# Autodesk Inventor assembly: ASY 000 ДМФ Disk Micro filter v3.0
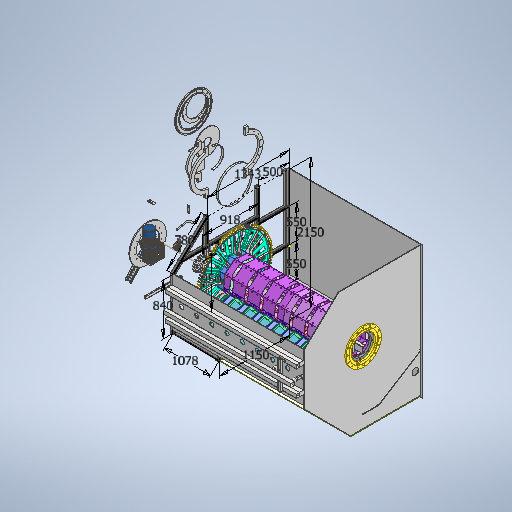
[picture p0: Inventor's stored thumbnail of the model, 512x512]
Saved by Autodesk Inventor 2026.2 (Build 302298000, 298)
## iProperties
Part Number: ASY 000 ДМФ Disk Micro filter v3.0
Document SubType Name: Assembly
Designer: admin
Author: admin
## Documents named in this file (43)
- C:\Users\admin\Documents\Inventor\DMF-Disk-Micro-Filter\ASY 000 ДМФ Disk Micro filter v3.0.iam
- C:\Users\admin\Documents\Inventor\DMF-Disk-Micro-Filter\Wall right v2.0.ipt
- C:\Users\admin\Documents\Inventor\DMF-Disk-Micro-Filter\DF1.03 Wall bottom v2.0.ipt
- C:\Users\admin\Documents\Inventor\DMF-Disk-Micro-Filter\DF1.04 Wall face v2.0.ipt
- C:\Users\admin\Documents\Inventor\DMF-Disk-Micro-Filter\ДМФ 021 кольцо прижимное нос v2.0.ipt
- C:\Users\admin\Documents\Inventor\DMF-Disk-Micro-Filter\ДМФ 032 крышка Нос v2.0.ipt
- C:\Users\admin\Documents\Inventor\DMF-Disk-Micro-Filter\ДМФ 091 Постель НОС v2.0.ipt
- C:\Users\admin\Documents\Inventor\DMF-Disk-Micro-Filter\ДМФ 022 кольцо прижимное корма v2.0.ipt
- C:\Users\admin\Documents\Inventor\DMF-Disk-Micro-Filter\ДМФ 093 Постель КОРМА v2.0.ipt
- C:\Users\admin\Documents\Inventor\DMF-Disk-Micro-Filter\ДМФ 092 Коромысло КОРМА v2.0.ipt
- C:\Users\admin\Documents\Inventor\DMF-Disk-Micro-Filter\ДМФ 055 труба илоотвода v2.0.ipt
- C:\Users\admin\Documents\Inventor\DMF-Disk-Micro-Filter\ДМФ 033 держатель лотка v2.0.ipt
- C:\Users\admin\Documents\Inventor\DMF-Disk-Micro-Filter\ASY ДМФ лоток 050 илоотвод v2.0.iam
- C:\Users\admin\Documents\Inventor\DMF-Disk-Micro-Filter\ДМФ 092 Коромысло НОС v2.0.ipt
- C:\Users\admin\Documents\Inventor\DMF-Disk-Micro-Filter\ДМФ 066 Гребенка v2.0.ipt
- C:\Users\admin\Documents\Inventor\DMF-Disk-Micro-Filter\ДМФ 025 кольцо прижимное корма наружное v2.0.ipt
- C:\Users\admin\Documents\Inventor\DMF-Disk-Micro-Filter\ДМФ 067 крышка v2.0.ipt
- C:\Users\admin\Documents\Inventor\DMF-Disk-Micro-Filter\ДМФ 081 труба форсунки v2.0.ipt
- C:\Users\admin\Documents\Inventor\DMF-Disk-Micro-Filter\ASY Обрешетка лицевая стенка.iam
- C:\Users\admin\Documents\Inventor\DMF-Disk-Micro-Filter\Вал ведущей шестерни.ipt
- C:\Users\admin\Documents\Inventor\DMF-Disk-Micro-Filter\Корпусный подшипник D35.ipt
- C:\Users\admin\Documents\Inventor\DMF-Disk-Micro-Filter\Мотор-редуктор NMRV 090(80B5).ipt
- C:\Users\admin\Documents\Inventor\DMF-Disk-Micro-Filter\DMF pancake.ipt
- C:\Users\admin\Documents\Inventor\DMF-Disk-Micro-Filter\Нога для постели.ipt
- C:\Users\admin\Documents\Inventor\DMF-Disk-Micro-Filter\Нога для постели №2.ipt
- C:\Users\admin\Documents\Inventor\DMF-Disk-Micro-Filter\ДМФ 092 Постель НОС v2.0.ipt
- C:\Users\admin\Documents\Inventor\DMF-Disk-Micro-Filter\ДМФ 094 Постель НОС крепление v2.0.ipt
- C:\Users\admin\Documents\Inventor\DMF-Disk-Micro-Filter\DMF Hat 2.0.ipt
- C:\Users\admin\Documents\Inventor\DMF-Disk-Micro-Filter\DMF Flange exit 2.0.ipt
- C:\Users\admin\Documents\Inventor\DMF-Disk-Micro-Filter\Барабан v2.1\ASY ДМФ 0100 Барабан v2.1.iam
- C:\Users\admin\Documents\Inventor\DMF-Disk-Micro-Filter\Барабан v2.1\DMF flange small gear.ipt
- C:\Users\admin\Documents\Inventor\DMF-Disk-Micro-Filter\Барабан v2.1\DMF small gear.ipt
- C:\Users\admin\Documents\Inventor\DMF-Disk-Micro-Filter\DMF Support ring tail.ipt
- C:\Users\admin\Documents\Inventor\DMF-Disk-Micro-Filter\DMF 082 коллектор болванка.ipt
- C:\Users\admin\Documents\Inventor\DMF-Disk-Micro-Filter\Барабан v2.1\DMF 2.1 Пластина паза маленькая.ipt
- C:\Users\admin\Documents\Inventor\DMF-Disk-Micro-Filter\Барабан v2.1\DMF 01 12 Барабан усилитель v2.1.ipt
- C:\Users\admin\Documents\Inventor\DMF-Disk-Micro-Filter\Барабан v2.1\DMF 2.1 01 45 Gear ring 5.ipt
- C:\Users\admin\Documents\Inventor\DMF-Disk-Micro-Filter\Барабан v2.1\DMF 2.1 01 46 Gear axis wheel 6.ipt
- C:\Users\admin\Documents\Inventor\DMF-Disk-Micro-Filter\Барабан v2.1\DMF 01 13 Барабан усилитель v2.1.ipt
- C:\Users\admin\Documents\Inventor\DMF-Disk-Micro-Filter\ДМФ 01 12 Барабан усилитель.ipt
- C:\Users\admin\Documents\Inventor\DMF-Disk-Micro-Filter\ДМФ 01 15 Барабан усилитель борта.ipt
- C:\Users\admin\Documents\Inventor\DMF-Disk-Micro-Filter\ДМФ 01 15 Барабан усилитель борта_CPY.ipt
- C:\Users\admin\Documents\Inventor\DMF-Disk-Micro-Filter\Барабан v2.1\DMF flange small gear 2.ipt
## Components (43 placed, 42 different names)
1. Wall right v2.0:1
2. DF1.03 Wall bottom v2.0:1
3. DF1.04 Wall face v2.0:1
4. ДМФ 021 кольцо прижимное нос v2.0:1
5. ДМФ 032 крышка Нос v2.0:1
6. ДМФ 091 Постель НОС v2.0:1
7. ДМФ 022 кольцо прижимное корма v2.0:1
8. ДМФ 093 Постель КОРМА v2.0:1
9. Постель 204 корма:1
10. ДМФ 055 труба илоотвода v2.0:1
11. ДМФ 033 держатель лотка v2.0:1
12. ASY ДМФ лоток 050 илоотвод v2.0:1 [sub-assembly]
13. ДМФ 092 Коромысло НОС v2.0:1
14. ДМФ 066 Гребенка v2.0:1
15. ДМФ 025 кольцо прижимное корма наружное v2.0:1
16. ДМФ 067 крышка v2.0:1
17. ДМФ 081 труба форсунки v2.0:1
18. ASY Обрешетка лицевая стенка:1 [sub-assembly]
19. Вал ведущей шестерни:1
20. Корпусный подшипник D35:1
21. Мотор-редуктор NMRV 090(80B5):1
22. DMF pancake:1
23. Нога для постели:1
24. Нога для постели №2:1
25. ДМФ 092 Постель НОС v2.0:1
26. ДМФ 094 Постель НОС крепление v2.0:1
27. DMF Hat 2.0:1
28. DMF Flange exit 2.0:1
29. ASY ДМФ 0100 Барабан v2.1:1 [sub-assembly]
30. flange small gear:1
31. DMF small gear:1
32. DMF Support ring tail:1
33. DMF 082 коллектор болванка:1
34. ДМФ 081 труба форсунки v2.0:2
35. DMF 2.1 Пластина паза маленькая:1
36. DMF 01 12 Барабан усилитель v2.1:1
37. DMF 2.1 01 45 Gear ring 5:1
38. DMF 2.1 01 46 Gear axis wheel 6:1
39. ДМФ 01 13 Барабан усилитель v2.0:1
40. ДМФ 01 12 Барабан усилитель:1
41. ДМФ 01 15 Барабан усилитель борта:1
42. ДМФ 01 15 Барабан усилитель борта_CPY:1
43. DMF flange small gear 2:1
## Relationships (25: Mate 9, WeldJoint 7, Flush 4, RevoluteJoint 3, Angle 1, CylindricalJoint 1)
- [Mate]: DF1.03 Wall bottom v2.0:1 ↔ DF1.04 Wall face v2.0:1
- [Angle] (180 deg): DF1.04 Wall face v2.0:1 ↔ ДМФ 066 Гребенка v2.0:1
- [Mate]: DF1.03 Wall bottom v2.0:1 ↔ ДМФ 066 Гребенка v2.0:1
- [Flush]: Wall right v2.0:1 ↔ ДМФ 067 крышка v2.0:1
- [WeldJoint]: ДМФ 055 труба илоотвода v2.0:1 ↔ DMF Flange exit 2.0:1
- [WeldJoint]: DMF pancake:1 ↔ DMF Hat 2.0:1
- [CylindricalJoint]: ДМФ 055 труба илоотвода v2.0:1 ↔ DMF Hat 2.0:1
- [WeldJoint]: Wall right v2.0:1 ↔ DMF Support ring tail:1
- [RevoluteJoint]: ASY ДМФ 0100 Барабан v2.1:1 ↔ DMF Support ring tail:1
- [RevoluteJoint]: ASY ДМФ 0100 Барабан v2.1:1 ↔ DMF Support ring tail:1
- [WeldJoint]: ДМФ 081 труба форсунки v2.0:1 ↔ DMF 082 коллектор болванка:1
- [WeldJoint]: DMF 082 коллектор болванка:1 ↔ ДМФ 081 труба форсунки v2.0:2
- [Mate]: Wall right v2.0:1 ↔ ДМФ 067 крышка v2.0:1
- [Mate] (40 mm): ДМФ 067 крышка v2.0:1 ↔ DMF 082 коллектор болванка:1
- [Mate]: DMF 082 коллектор болванка:1 ↔ ДМФ 01 15 Барабан усилитель борта:1
- [Mate]: DMF 082 коллектор болванка:1 ↔ ДМФ 01 15 Барабан усилитель борта:1
- [Flush]: ДМФ 067 крышка v2.0:1 ↔ DMF 082 коллектор болванка:1
- [Mate]: ДМФ 033 держатель лотка v2.0:1 ↔ ДМФ 067 крышка v2.0:1
- [Mate]: ДМФ 067 крышка v2.0:1 ↔ ДМФ 01 15 Барабан усилитель борта_CPY:1
- [Flush]: ДМФ 033 держатель лотка v2.0:1 ↔ ДМФ 01 15 Барабан усилитель борта_CPY:1
- [RevoluteJoint]: Вал ведущей шестерни:1 ↔ DMF small gear:1
- [WeldJoint]: flange small gear:1 ↔ DMF flange small gear 2:1
- [WeldJoint] (-25 mm): Вал ведущей шестерни:1 ↔ flange small gear:1
- [Flush]: ASY Обрешетка лицевая стенка:1 ↔ Нога для постели №2:1
- [Mate]: ASY Обрешетка лицевая стенка:1 ↔ Нога для постели №2:1
